# Autodesk Inventor assembly: Falcon_500_Powered_by_Talon_FX_217-6515
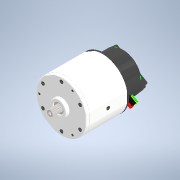
[picture p0: Inventor's stored thumbnail of the model, 180x180]
Saved by Autodesk Inventor 2020 (Build 240168000, 168)
## iProperties
Created: 2019-10-30
Part Number: Falcon_500_Powered_by_Talon_FX_217-6515
Description: STEP AP214
Document SubType Name: Assembly
Designer: srini
Sending System: SolidWorks 2017
Preprocessor: SwSTEP 2.0
Title: 217-6515 20190920.STEP
Revision Number: ANY
## Documents named in this file (13)
- C:\Users\srini\Documents\FRC\2020\Shooter\Falcon_500_Powered_by_Talon_FX_217-6515.iam
- C:\Users\srini\Documents\FRC\2020\Shooter\217-6515-Back 20190920.ipt
- C:\Users\srini\Documents\FRC\2020\Shooter\217-6515-002 Rev6.ipt
- C:\Users\srini\Documents\FRC\2020\Shooter\M2.5 SHCS, Grade 8 Steel Rev1_SSAM2.5-06MMZB.ipt
- C:\Users\srini\Documents\FRC\2020\Shooter\217-6515-010 Rev1_9262K442.ipt
- C:\Users\srini\Documents\FRC\2020\Shooter\217-6515-001 Rev6.ipt
- C:\Users\srini\Documents\FRC\2020\Shooter\217-6515-005 Rev4_7804K116.ipt
- C:\Users\srini\Documents\FRC\2020\Shooter\M3 BHTS-SECURE, Grade 8 Steel Rev1_SBTM3-24MMZB-SECURE.ipt
- C:\Users\srini\Documents\FRC\2020\Shooter\M3 BHTS, Grade 8 Steel Rev1_SBTM3-50MMZB.ipt
- C:\Users\srini\Documents\FRC\2020\Shooter\217-6515-308 Rev5.ipt
- C:\Users\srini\Documents\FRC\2020\Shooter\#4-40 SHCS, Grade 8 Steel Rev2_SSA0440-0125ZB.ipt
- C:\Users\srini\Documents\FRC\2020\Shooter\217-4649-007 Rev1_94105A824.ipt
- C:\Users\srini\Documents\FRC\2020\Shooter\Falcon_Motor_Short_Shaft_217-6958.iam
## Components (27 placed, 27 different names)
1. 217-6515-Back 20190920_1 — Insert:1
2. 217-6515-002 Rev6_3 — Insert:2
3. M2.5 SHCS, Grade 8 Steel Rev1_SSAM2.5-06MMZB_4
4. M2.5 SHCS, Grade 8 Steel Rev1_SSAM2.5-06MMZB_5 — Mate:1
5. M2.5 SHCS, Grade 8 Steel Rev1_SSAM2.5-06MMZB_6
6. M2.5 SHCS, Grade 8 Steel Rev1_SSAM2.5-06MMZB_7
7. M2.5 SHCS, Grade 8 Steel Rev1_SSAM2.5-06MMZB_8
8. 217-6515-010 Rev1_9262K442_9
9. 217-6515-001 Rev6_10 — Insert:2
10. 217-6515-005 Rev4_7804K116_11
11. M3 BHTS-SECURE, Grade 8 Steel Rev1_SBTM3-24MMZB-SECURE_12
12. M3 BHTS-SECURE, Grade 8 Steel Rev1_SBTM3-24MMZB-SECURE_13
13. M3 BHTS-SECURE, Grade 8 Steel Rev1_SBTM3-24MMZB-SECURE_14
14. M3 BHTS, Grade 8 Steel Rev1_SBTM3-50MMZB_15
15. M3 BHTS, Grade 8 Steel Rev1_SBTM3-50MMZB_16
16. M3 BHTS, Grade 8 Steel Rev1_SBTM3-50MMZB_17
17. 217-6515-308 Rev5_18
18. #4-40 SHCS, Grade 8 Steel Rev2_SSA0440-0125ZB_19
19. #4-40 SHCS, Grade 8 Steel Rev2_SSA0440-0125ZB_20
20. 217-4649-007 Rev1_94105A824_21
21. 217-4649-007 Rev1_94105A824_22
22. 217-4649-007 Rev1_94105A824_23
23. 217-4649-007 Rev1_94105A824_24
24. 217-4649-007 Rev1_94105A824_25
25. 217-4649-007 Rev1_94105A824_26
26. 217-4649-007 Rev1_94105A824_27
27. Falcon_Motor_Short_Shaft_217-6958:1 [sub-assembly] — Insert:1, Mate:1
## Relationships (3: Insert 2, Mate 1)
- Insert:1: 217-6515-Back 20190920_1 ↔ Falcon_Motor_Short_Shaft_217-6958:1
- Mate:1: M2.5 SHCS, Grade 8 Steel Rev1_SSAM2.5-06MMZB_5 ↔ Falcon_Motor_Short_Shaft_217-6958:1
- Insert:2: 217-6515-002 Rev6_3 ↔ 217-6515-001 Rev6_10
